# Autodesk Inventor assembly: Hotend Mount Assembly_MIR3
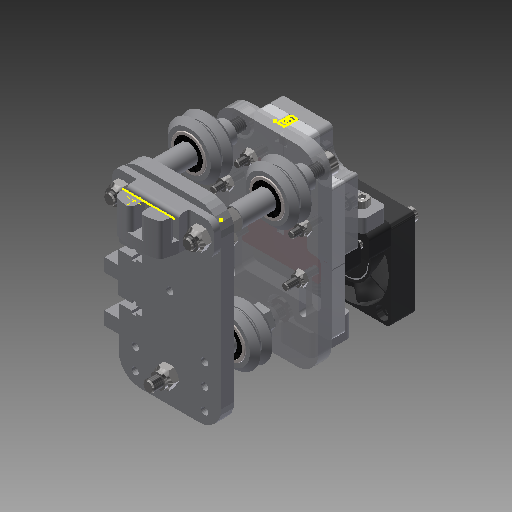
[picture p0: Inventor's stored thumbnail of the model, 512x512]
Saved by Autodesk Inventor 2017 (Build 210142000, 142)
## iProperties
Created: 2016-06-23
Part Number: Hotend Mount Assembly_MIR3
Document SubType Name: Assembly
Designer: User
Author: joshmamo
## Documents named in this file (24)
- C:\All INVENTOR\SL-Inventor\SL-Beast 3D Printer\Hotend Mount Assembly_MIR3.iam
- C:\All INVENTOR\SL-Inventor\SL-Beast 3D Printer\Hotend Slide Part 1_MIR3.ipt
- C:\All INVENTOR\SL-Inventor\SL-Beast 3D Printer\Hotend Slide Part 2_MIR3.ipt
- C:\All INVENTOR\SL-Inventor\SL-Beast 3D Printer\Hotend Slide Part3_MIR3.ipt
- C:\All INVENTOR\SL-Inventor\SL-Beast 3D Printer\Hotend Front Plate revised_MIR3.ipt
- C:\All INVENTOR\SL-Inventor\SL-Beast 3D Printer\Working Axis etc_MIR3.ipt
- C:\All INVENTOR\SL-Inventor\SL-Beast 3D Printer\Hotend Clamp P1_MIR3.ipt
- C:\All INVENTOR\SL-Inventor\SL-Beast 3D Printer\Hotend Clamp P2_MIR3.ipt
- C:\All INVENTOR\SL-Inventor\SL-Beast 3D Printer\Hotend Mock Up_MIR3.ipt
- C:\All INVENTOR\SL-Inventor\SL-Beast 3D Printer\en-US\ANSI B18.3.1M(6)\ANSI B18.3.1M - M3x0.5 x 25(1).ipt
- C:\All INVENTOR\SL-Inventor\SL-Beast 3D Printer\R2017\en-US\ANSI B18.3.1M(6)\ANSI B18.3.1M - M3x0.5 x 30(1).ipt
- C:\All INVENTOR\SL-Inventor\SL-Beast 3D Printer\R2017\en-US\AS 1474(2)\AS 1474 - M3(2).ipt
- C:\All INVENTOR\SL-Inventor\SL-Beast 3D Printer\pshfit-mount-acrylic_MIR3.ipt
- C:\All INVENTOR\SL-Inventor\SL-Beast 3D Printer\en-US\ANSI B18.3.1M(6)\ANSI B18.3.1M - M3x0.5 x 20(1).ipt
- C:\All INVENTOR\SL-Inventor\SL-Beast 3D Printer\R2017\en-US\ANSI B 18.2.4.1 M(1)\ANSI B 18.2.4.1 M - M3 x 0.5Style 2.ipt
- C:\All INVENTOR\SL-Inventor\SL-Beast 3D Printer\Pushfit-Adapter_MIR3.iam
- C:\All INVENTOR\SL-Inventor\SL-Beast 3D Printer\en-US\ANSI B18.16.3M(2)\ANSI B18.16.3M - Property Class 5 and 10 - Metric M3 x 0.5 Metal Type.ipt
- C:\All INVENTOR\SL-Inventor\SL-Beast 3D Printer\40mm_fan_MIR3.ipt
- C:\All INVENTOR\SL-Inventor\SL-Beast 3D Printer\R2017\en-US\ANSI B18.3.1M(6)\ANSI B18.3.1M - M3x0.5 x 55(1).ipt
- C:\All INVENTOR\SL-Inventor\SL-Beast 3D Printer\DelrinX-Wheel-Top_MIR3.iam
- C:\All INVENTOR\SL-Inventor\SL-Beast 3D Printer\DelrinX-Wheel-Bottom_MIR3.iam
- C:\All INVENTOR\SL-Inventor\SL-Beast 3D Printer\Hotend Rear Plate_MIR3.ipt
- C:\All INVENTOR\SL-Inventor\SL-Beast 3D Printer\en-US\ANSI B18.16.3M(2)\ANSI B18.16.3M - Property Class 9 - Metric M5 x 0.8 Metal Type.ipt
- C:\All INVENTOR\SL-Inventor\SL-Beast 3D Printer\X Belt Holder_MIR3.iam
## Components (37 placed, 23 different names)
1. Hotend Slide Part 1_MIR3:1
2. Hotend Slide Part 2_MIR3:1
3. Hotend Slide Part3_MIR3:1
4. Hotend Front Plate revised_MIR3:1 — Insert:5, Insert:7, Insert:8, Insert:10, Insert:11, Insert:12, Mate:15, Mate:13, Mate:16, Mate:14, Mate:18, Mate:17, Flush:6, Flush:5, Flush:4
5. Working Axis etc_MIR3:1
6. Hotend Clamp P1_MIR3:1 — Flush:2, Mate:1, Flush:1
7. Hotend Clamp P2_MIR3:1 — Flush:2, Mate:1, Flush:1, Mate:4, Mate:2, Mate:6, Mate:8, Mate:12, Mate:11
8. Hotend Mock Up_MIR3:1 — Mate:3
9. Forged Socket Head Cap Screw - Metric M3x0.5 x 25:1
10. Forged Socket Head Cap Screw - Metric M3x0.5 x 25:2
11. Forged Socket Head Cap Screw - Metric M3x0.5 x 25:3
12. Forged Socket Head Cap Screw - Metric M3x0.5 x 25:4
13. Forged Socket Head Cap Screw - Metric M3x0.5 x 30:1
14. AS 1474 (Square Nut) - Metric M3:1
15. pshfit-mount-acrylic_MIR3:1 — Mate:4, Mate:3, Mate:2, Insert:1, Insert:2, Mate:10, Mate:9
16. Forged Socket Head Cap Screw - Metric M3x0.5 x 20:1 — Insert:1, Mate:5
17. Forged Socket Head Cap Screw - Metric M3x0.5 x 20:2 — Insert:2, Mate:7
18. Hex Nut Metric M3 x 0.5:1 — Mate:6, Mate:5
19. Hex Nut Metric M3 x 0.5:2 — Mate:8, Mate:7
20. Pushfit-Adapter_MIR3:1 [sub-assembly] — Mate:10, Mate:9
21. Prevailing Torque Type Hex Nut - Steel Metric Property Class 5 and 10 - Metric M3 x 0.5 Metal Type:1 — Insert:5
22. Prevailing Torque Type Hex Nut - Steel Metric Property Class 5 and 10 - Metric M3 x 0.5 Metal Type:2 — Insert:7
23. Prevailing Torque Type Hex Nut - Steel Metric Property Class 5 and 10 - Metric M3 x 0.5 Metal Type:3 — Insert:8
24. Prevailing Torque Type Hex Nut - Steel Metric Property Class 5 and 10 - Metric M3 x 0.5 Metal Type:4 — Insert:10
25. Prevailing Torque Type Hex Nut - Steel Metric Property Class 5 and 10 - Metric M3 x 0.5 Metal Type:5 — Insert:11
26. Prevailing Torque Type Hex Nut - Steel Metric Property Class 5 and 10 - Metric M3 x 0.5 Metal Type:6 — Insert:12
27. 40mm_fan_MIR3:1 — Mate:12, Mate:11, Insert:13, Insert:16
28. Forged Socket Head Cap Screw - Metric M3x0.5 x 55:1 — Insert:13
29. Forged Socket Head Cap Screw - Metric M3x0.5 x 55:2 — Insert:16
30. DelrinX-Wheel-Top_MIR3:1 [sub-assembly] — Mate:15, Mate:13, Mate:26, Mate:27
31. DelrinX-Wheel-Top_MIR3:2 [sub-assembly] — Mate:16, Mate:14, Mate:29
32. DelrinX-Wheel-Bottom_MIR3:1 [sub-assembly] — Mate:18, Mate:17, Mate:23
33. Hotend Rear Plate_MIR3:1 — Flush:6, Flush:5, Flush:4, Mate:24, Angle:1, Mate:25
34. Prevailing Torque Type Hex Nut - Steel Metric Property Class 9 - Metric M5 x 0.8 Metal Type:1 — Mate:24, Mate:23
35. X Belt Holder_MIR3:1 [sub-assembly] — Mate:26, Angle:1, Mate:25, Mate:28, Mate:30
36. Prevailing Torque Type Hex Nut - Steel Metric Property Class 9 - Metric M5 x 0.8 Metal Type:2 — Mate:28, Mate:27
37. Prevailing Torque Type Hex Nut - Steel Metric Property Class 9 - Metric M5 x 0.8 Metal Type:3 — Mate:30, Mate:29
## Relationships (42: Mate 26, Insert 10, Flush 5, Angle 1)
- Flush:2: Hotend Clamp P1_MIR3:1 ↔ Hotend Clamp P2_MIR3:1
- Mate:1 (4 mm): Hotend Clamp P1_MIR3:1 ↔ Hotend Clamp P2_MIR3:1
- Flush:1: Hotend Clamp P1_MIR3:1 ↔ Hotend Clamp P2_MIR3:1
- Mate:4: Hotend Clamp P2_MIR3:1 ↔ pshfit-mount-acrylic_MIR3:1
- Mate:3: Hotend Mock Up_MIR3:1 ↔ pshfit-mount-acrylic_MIR3:1
- Mate:2: Hotend Clamp P2_MIR3:1 ↔ pshfit-mount-acrylic_MIR3:1
- Insert:1: pshfit-mount-acrylic_MIR3:1 ↔ Forged Socket Head Cap Screw - Metric M3x0.5 x 20:1
- Insert:2: pshfit-mount-acrylic_MIR3:1 ↔ Forged Socket Head Cap Screw - Metric M3x0.5 x 20:2
- Mate:6: Hotend Clamp P2_MIR3:1 ↔ Hex Nut Metric M3 x 0.5:1
- Mate:5: Forged Socket Head Cap Screw - Metric M3x0.5 x 20:1 ↔ Hex Nut Metric M3 x 0.5:1
- Mate:8: Hotend Clamp P2_MIR3:1 ↔ Hex Nut Metric M3 x 0.5:2
- Mate:7: Forged Socket Head Cap Screw - Metric M3x0.5 x 20:2 ↔ Hex Nut Metric M3 x 0.5:2
- Mate:10: pshfit-mount-acrylic_MIR3:1 ↔ Pushfit-Adapter_MIR3:1
- Mate:9: pshfit-mount-acrylic_MIR3:1 ↔ Pushfit-Adapter_MIR3:1
- Insert:5: Hotend Front Plate revised_MIR3:1 ↔ Prevailing Torque Type Hex Nut - Steel Metric Property Class 5 and 10 - Metric M3 x 0.5 Metal Type:1
- Insert:7: Hotend Front Plate revised_MIR3:1 ↔ Prevailing Torque Type Hex Nut - Steel Metric Property Class 5 and 10 - Metric M3 x 0.5 Metal Type:2
- Insert:8: Hotend Front Plate revised_MIR3:1 ↔ Prevailing Torque Type Hex Nut - Steel Metric Property Class 5 and 10 - Metric M3 x 0.5 Metal Type:3
- Insert:10: Hotend Front Plate revised_MIR3:1 ↔ Prevailing Torque Type Hex Nut - Steel Metric Property Class 5 and 10 - Metric M3 x 0.5 Metal Type:4
- Insert:11: Hotend Front Plate revised_MIR3:1 ↔ Prevailing Torque Type Hex Nut - Steel Metric Property Class 5 and 10 - Metric M3 x 0.5 Metal Type:5
- Insert:12: Hotend Front Plate revised_MIR3:1 ↔ Prevailing Torque Type Hex Nut - Steel Metric Property Class 5 and 10 - Metric M3 x 0.5 Metal Type:6
- Mate:12: Hotend Clamp P2_MIR3:1 ↔ 40mm_fan_MIR3:1
- Mate:11: Hotend Clamp P2_MIR3:1 ↔ 40mm_fan_MIR3:1
- Insert:13: 40mm_fan_MIR3:1 ↔ Forged Socket Head Cap Screw - Metric M3x0.5 x 55:1
- Insert:16: 40mm_fan_MIR3:1 ↔ Forged Socket Head Cap Screw - Metric M3x0.5 x 55:2
- Mate:15: Hotend Front Plate revised_MIR3:1 ↔ DelrinX-Wheel-Top_MIR3:1
- Mate:13: Hotend Front Plate revised_MIR3:1 ↔ DelrinX-Wheel-Top_MIR3:1
- Mate:16: Hotend Front Plate revised_MIR3:1 ↔ DelrinX-Wheel-Top_MIR3:2
- Mate:14: Hotend Front Plate revised_MIR3:1 ↔ DelrinX-Wheel-Top_MIR3:2
- Mate:18: Hotend Front Plate revised_MIR3:1 ↔ DelrinX-Wheel-Bottom_MIR3:1
- Mate:17: Hotend Front Plate revised_MIR3:1 ↔ DelrinX-Wheel-Bottom_MIR3:1
- Flush:6: Hotend Front Plate revised_MIR3:1 ↔ Hotend Rear Plate_MIR3:1
- Flush:5: Hotend Front Plate revised_MIR3:1 ↔ Hotend Rear Plate_MIR3:1
- Flush:4: Hotend Front Plate revised_MIR3:1 ↔ Hotend Rear Plate_MIR3:1
- Mate:24: Hotend Rear Plate_MIR3:1 ↔ Prevailing Torque Type Hex Nut - Steel Metric Property Class 9 - Metric M5 x 0.8 Metal Type:1
- Mate:23: DelrinX-Wheel-Bottom_MIR3:1 ↔ Prevailing Torque Type Hex Nut - Steel Metric Property Class 9 - Metric M5 x 0.8 Metal Type:1
- Mate:26: DelrinX-Wheel-Top_MIR3:1 ↔ X Belt Holder_MIR3:1
- Angle:1 (0 deg): Hotend Rear Plate_MIR3:1 ↔ X Belt Holder_MIR3:1
- Mate:25: Hotend Rear Plate_MIR3:1 ↔ X Belt Holder_MIR3:1
- Mate:28: X Belt Holder_MIR3:1 ↔ Prevailing Torque Type Hex Nut - Steel Metric Property Class 9 - Metric M5 x 0.8 Metal Type:2
- Mate:27: DelrinX-Wheel-Top_MIR3:1 ↔ Prevailing Torque Type Hex Nut - Steel Metric Property Class 9 - Metric M5 x 0.8 Metal Type:2
- Mate:30: X Belt Holder_MIR3:1 ↔ Prevailing Torque Type Hex Nut - Steel Metric Property Class 9 - Metric M5 x 0.8 Metal Type:3
- Mate:29: DelrinX-Wheel-Top_MIR3:2 ↔ Prevailing Torque Type Hex Nut - Steel Metric Property Class 9 - Metric M5 x 0.8 Metal Type:3
